# Autodesk Inventor assembly: Parallel Axis Assembly
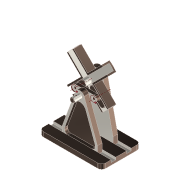
[picture p0: Inventor's stored thumbnail of the model, 180x180]
Saved by Autodesk Inventor 2022.2 (Build 262287010, 287A)
## iProperties
Created: 2022-12-29
Part Number: Parallel Axis Assembly
Document SubType Name: Assembly
Designer: User
Author: User
## Documents named in this file (8)
- C:\Users\User\Desktop\InventorTutorial prof Stancesu\Part19 Parallel axis coupling\Parallel Axis Assembly.iam
- C:\Users\User\Desktop\InventorTutorial prof Stancesu\Part19 Parallel axis coupling\Parallel axis parts\Plate.ipt
- C:\Users\User\Desktop\InventorTutorial prof Stancesu\Part19 Parallel axis coupling\Parallel axis parts\Axle.ipt
- C:\Users\User\Desktop\InventorTutorial prof Stancesu\Part19 Parallel axis coupling\Parallel axis parts\Bearing High.ipt
- C:\Users\User\Desktop\InventorTutorial prof Stancesu\Part19 Parallel axis coupling\Parallel axis parts\Bearing Short.ipt
- C:\Users\User\Desktop\InventorTutorial prof Stancesu\Part19 Parallel axis coupling\Parallel axis parts\Cross.ipt
- C:\Users\User\Desktop\InventorTutorial prof Stancesu\Part19 Parallel axis coupling\Parallel axis parts\Crank.ipt
- C:\Users\User\Desktop\InventorTutorial prof Stancesu\Part19 Parallel axis coupling\Parallel axis parts\Slider.ipt
## Components (9 placed, 7 different names)
1. Plate:1 — Mate:1, Mate:2, Mate:4, Mate:5, Angle:1
2. Axle:1 — Insert:1
3. Axle:2 — Insert:2
4. Bearing High:1 — Mate:1, Mate:2, Insert:6, Mate:3
5. Bearing Short:1 — Insert:5, Mate:4, Mate:5, Mate:6
6. Cross:1 — Insert:6, Mate:7, Mate:8
7. Crank:1 — Insert:3, Insert:4, Insert:5, Angle:1
8. Slider:1 — Insert:1, Insert:3, Mate:7
9. Slider:2 — Insert:2, Insert:4, Mate:8
## Relationships (15: Mate 8, Insert 6, Angle 1)
- Insert:1: Axle:1 ↔ Slider:1
- Insert:2: Axle:2 ↔ Slider:2
- Insert:3: Crank:1 ↔ Slider:1
- Insert:4: Crank:1 ↔ Slider:2
- Insert:5: Bearing Short:1 ↔ Crank:1
- Mate:1: Plate:1 ↔ Bearing High:1
- Mate:2: Plate:1 ↔ Bearing High:1
- Insert:6: Bearing High:1 ↔ Cross:1
- Mate:3: Bearing High:1
- Mate:4: Plate:1 ↔ Bearing Short:1
- Mate:5: Plate:1 ↔ Bearing Short:1
- Mate:6: Bearing Short:1
- Mate:7: Cross:1 ↔ Slider:1
- Mate:8: Cross:1 ↔ Slider:2
- Angle:1 (0 deg): Plate:1 ↔ Crank:1
